# Autodesk Inventor assembly: 212
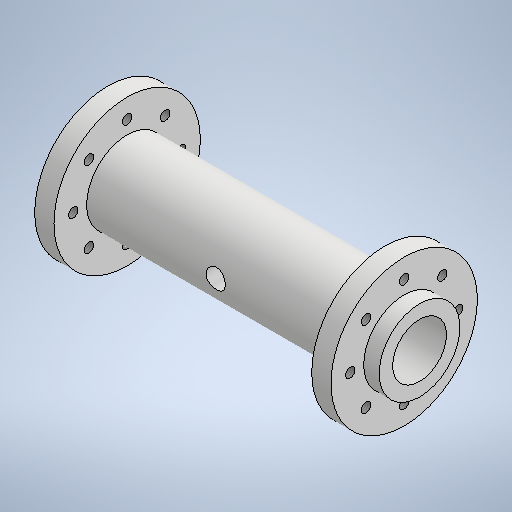
[picture p0: Inventor's stored thumbnail of the model, 512x512]
Saved by Autodesk Inventor 2025 (Build 290162010, 162A)
## iProperties
Created: 2024-06-09
Part Number: 212
Document SubType Name: Assembly
Designer: Fabri
Author: Fabri
## Documents named in this file (3)
- C:\Users\Fabri\Documents\Inventor\Paddle\212.iam
- C:\Users\Fabri\Documents\Inventor\Paddle\212.ipt
- C:\Users\Fabri\Documents\Inventor\Paddle\212.1.ipt
## Components (3 placed, 2 different names)
1. 212:1 — Insert:2
2. 212:2 — Insert:1
3. 212.1:1 — Insert:1, Insert:2
## Relationships (2: Insert 2)
- Insert:1 (-9 mm): 212:2 ↔ 212.1:1
- Insert:2 (-9 mm): 212:1 ↔ 212.1:1
